# Autodesk Inventor assembly: 95650
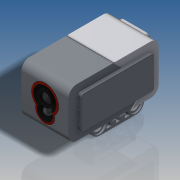
[picture p0: Inventor's stored thumbnail of the model, 180x180]
Saved by Autodesk Inventor 2016 SP2 (Build 200236200, 236)
## iProperties
Created: 2015-08-28
Part Number: 95650
Document SubType Name: Assembly
Designer: D. Kohfeld
Mass: 11.1836 g
Surface Area: 167.039 cm^2
Volume: 10.5294 cm^3
Density: 1.06213 g/cm^3
Author: D. Kohfeld
## Documents named in this file (8)
- A:\LEGO Pieces\EV3\95650.iam
- A:\LEGO Pieces\EV3\99377-LtBluishGray.ipt
- A:\LEGO Pieces\EV3\54732b-LtBluishGray.ipt
- A:\LEGO Pieces\EV3\99376-White.ipt
- A:\LEGO Pieces\EV3\11013-TransClear.ipt
- A:\LEGO Pieces\EV3\99396-TransClear.ipt
- A:\LEGO Pieces\EV3\11014p01-Black.ipt
- A:\LEGO Pieces\EV3\99388-LtBluishGray.ipt
## Components (7 placed, 7 different names)
1. 99377-LtBluishGray:1 — Flush:1, Mate:3, Mate:4, Flush:2, Flush:4, Mate:6, Mate:7
2. 54732b-LtBluishGray:1 — Mate:7, Flush:6, Mate:8
3. 99376-White:1 — Flush:4, Flush:5, Mate:6, Flush:6, Mate:8
4. 11013-TransClear:1 — Angle:1, Mate:1, Tangent:1
5. 99396-TransClear:1 — Angle:2, Mate:2, Tangent:2
6. 11014p01-Black:1 — Angle:1, Angle:2, Mate:1, Mate:2, Tangent:1, Tangent:2, Flush:2, Mate:5, Flush:3
7. 99388-LtBluishGray:1 — Flush:1, Mate:3, Mate:4, Mate:5, Flush:3, Flush:5
## Relationships (18: Mate 8, Flush 6, Angle 2, Tangent 2)
- Angle:1 (0 deg): 11013-TransClear:1 ↔ 11014p01-Black:1
- Angle:2 (0 deg): 99396-TransClear:1 ↔ 11014p01-Black:1
- Mate:1: 11013-TransClear:1 ↔ 11014p01-Black:1
- Mate:2: 99396-TransClear:1 ↔ 11014p01-Black:1
- Tangent:1: 11013-TransClear:1 ↔ 11014p01-Black:1
- Tangent:2: 99396-TransClear:1 ↔ 11014p01-Black:1
- Flush:1: 99377-LtBluishGray:1 ↔ 99388-LtBluishGray:1
- Mate:3: 99377-LtBluishGray:1 ↔ 99388-LtBluishGray:1
- Mate:4: 99377-LtBluishGray:1 ↔ 99388-LtBluishGray:1
- Flush:2: 99377-LtBluishGray:1 ↔ 11014p01-Black:1
- Mate:5: 11014p01-Black:1 ↔ 99388-LtBluishGray:1
- Flush:3: 11014p01-Black:1 ↔ 99388-LtBluishGray:1
- Flush:4: 99377-LtBluishGray:1 ↔ 99376-White:1
- Flush:5: 99376-White:1 ↔ 99388-LtBluishGray:1
- Mate:6: 99377-LtBluishGray:1 ↔ 99376-White:1
- Mate:7: 99377-LtBluishGray:1 ↔ 54732b-LtBluishGray:1
- Flush:6: 54732b-LtBluishGray:1 ↔ 99376-White:1
- Mate:8: 54732b-LtBluishGray:1 ↔ 99376-White:1
